# Autodesk Inventor assembly: Assembly_v2
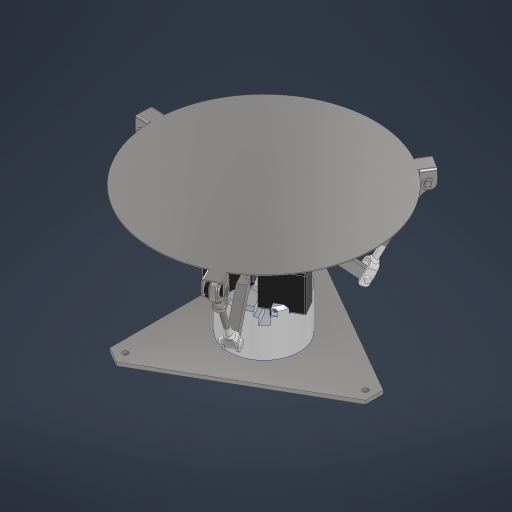
[picture p0: Inventor's stored thumbnail of the model, 512x512]
Saved by Autodesk Inventor 2023 (Build 270158000, 158)
## iProperties
Created: 2023-02-25
Part Number: Assembly_v2
Document SubType Name: Assembly
Designer: roota
Mass: 2505.51 g
Surface Area: 3613.46 cm^2
Volume: 474.073 cm^3
Density: 5.28507 g/cm^3
Author: roota
## Documents named in this file (18)
- D:\GitHub\NTUST-Mechanical-Design\Ball stabilization mechanism\3D CAD files\Mechanical Part CAD files\Assemblies\Assembly_v2.iam
- D:\GitHub\NTUST-Mechanical-Design\Ball stabilization mechanism\3D CAD files\Mechanical Part CAD files\Static Mechanisms\BasePlate.ipt
- D:\GitHub\NTUST-Mechanical-Design\Ball stabilization mechanism\3D CAD files\Mechanical Part CAD files\Static Mechanisms\BaseSupport.ipt
- D:\GitHub\NTUST-Mechanical-Design\Ball stabilization mechanism\3D CAD files\Electrical Hardware CAD files\SERVO\LDX-335MG_Servo_15kg_cm.ipt
- D:\GitHub\NTUST-Mechanical-Design\Ball stabilization mechanism\3D CAD files\Mechanical Part CAD files\Static Mechanisms\ServoCap V2.ipt
- C:\Users\roota\Documents\Inventor\Content Center Files\R2023\en-US\ISO 10642(2)\ISO 10642  - M8  x  80.ipt
- C:\Users\roota\Documents\Inventor\Content Center Files\R2023\en-US\ISO 10642(2)\ISO 10642  - M5  x  12.ipt
- C:\Users\roota\Documents\Inventor\Content Center Files\R2023\en-US\ISO 4762(2)\ISO 4762 - M5 x 12ISO.ipt
- C:\Users\roota\Documents\Inventor\Content Center Files\R2023\en-US\BS EN ISO 4026\BS EN ISO 4168 - M3 x 6(2).ipt
- D:\GitHub\NTUST-Mechanical-Design\Ball stabilization mechanism\3D CAD files\Electrical Hardware CAD files\SERVO\ServoDrive.ipt
- D:\GitHub\NTUST-Mechanical-Design\Ball stabilization mechanism\3D CAD files\Mechanical Part CAD files\Dynamic Mechanisms\Servo_Strut_v2.ipt
- D:\GitHub\NTUST-Mechanical-Design\Ball stabilization mechanism\3D CAD files\Mechanical Part CAD files\Hardware Parts\M6x1 Welded thread fork\M6x1 Welded thread fork.ipt
- D:\GitHub\NTUST-Mechanical-Design\Ball stabilization mechanism\3D CAD files\Mechanical Part CAD files\Hardware Parts\SELF-LUBRIFICATING ROD END\End_6mm.ipt
- D:\GitHub\NTUST-Mechanical-Design\Ball stabilization mechanism\3D CAD files\Mechanical Part CAD files\Hardware Parts\SELF-LUBRIFICATING ROD END\Ball_6mm_male.ipt
- D:\GitHub\NTUST-Mechanical-Design\Ball stabilization mechanism\3D CAD files\Mechanical Part CAD files\Static Mechanisms\rod pin.ipt
- C:\Users\roota\Documents\Inventor\Content Center Files\R2023\en-US\JIS B 2804 E\_JIS B 2804 E - 5 - 6.ipt
- D:\GitHub\NTUST-Mechanical-Design\Ball stabilization mechanism\3D CAD files\Mechanical Part CAD files\Static Mechanisms\4mm spacer.ipt
- D:\GitHub\NTUST-Mechanical-Design\Ball stabilization mechanism\3D CAD files\Mechanical Part CAD files\Static Mechanisms\BalancePlate.ipt
## Components (51 placed, 17 different names)
1. BasePlate:1 — Mate:46, Mate:47, Mate:48, Mate:49, Mate:50, Mate:51, Mate:63, Mate:64, Mate:65, Mate:66
2. BaseSupport:1 — Mate:49, Mate:50, Mate:51, Mate:52, Mate:53, Mate:54, Mate:55, Mate:56, Mate:57, Mate:58, Mate:59, Mate:60, Mate:67, Mate:68, Mate:69
3. LDX-335MG_Servo_15kg_cm:1 — Mate:52, Mate:53, Mate:54, Mate:61, Insert:1, Insert:2, Insert:9
4. LDX-335MG_Servo_15kg_cm:2 — Mate:55, Mate:59, Mate:60, Insert:3, Insert:4, Insert:7
5. LDX-335MG_Servo_15kg_cm:3 — Mate:56, Mate:57, Mate:58, Insert:5, Insert:6, Insert:8
6. ServoCap V2:1 — Mate:61, Mate:62, Mate:70, Mate:82
7. DIN EN ISO 10642 M8  x  80:1 — Mate:62
8. DIN EN ISO 10642 M5  x  12:1 — Mate:63
9. DIN EN ISO 10642 M5  x  12:2 — Mate:64
10. DIN EN ISO 10642 M5  x  12:3 — Mate:65
11. DIN EN ISO 10642 M5  x  12:4 — Mate:66
12. ISO 4762 M5 x 12:1 — Insert:1
13. ISO 4762 M5 x 12:2 — Insert:2
14. ISO 4762 M5 x 12:3 — Insert:3
15. ISO 4762 M5 x 12:4 — Insert:4, Mate:70
16. ISO 4762 M5 x 12:5 — Insert:5
17. ISO 4762 M5 x 12:6 — Insert:6
18. BS EN ISO 4026 - Metric M3 x 6:1 — Mate:67
19. BS EN ISO 4026 - Metric M3 x 6:2 — Mate:68
20. BS EN ISO 4026 - Metric M3 x 6:3 — Mate:69
21. ServoDrive:1 — Insert:7, Insert:10
22. ServoDrive:2 — Insert:8, Insert:11
23. ServoDrive:3 — Insert:9, Insert:12
24. Servo_Strut_v2:1 — Insert:10, Insert:13
25. Servo_Strut_v2:2 — Insert:11, Insert:14
26. Servo_Strut_v2:3 — Insert:12, Insert:15
27. M6x1 Welded thread fork:1 — Insert:13, Insert:16, Angle:1
28. M6x1 Welded thread fork:2 — Insert:14, Insert:18, Angle:2
29. M6x1 Welded thread fork:3 — Insert:15, Insert:17, Angle:3
30. End_6mm:1 — Insert:16, Angle:1, Tangent:3
31. End_6mm:2 — Insert:17, Angle:3, Tangent:1
32. End_6mm:3 — Insert:18, Angle:2, Tangent:2
33. Ball_6mm_male:1 — Tangent:1, Insert:25, Insert:26
34. Ball_6mm_male:2 — Tangent:2, Insert:29, Insert:30
35. Ball_6mm_male:3 — Tangent:3, Insert:27, Insert:28
36. rod pin:1 — Insert:23, Insert:24, Mate:71, Mate:74
37. rod pin:2 — Insert:19, Insert:20, Mate:72
38. rod pin:3 — Insert:21, Insert:22, Mate:73
39. JIS B 2804 E 5:1 — Insert:19
40. JIS B 2804 E 5:2 — Insert:20, Mate:78
41. JIS B 2804 E 5:3 — Insert:21, Mate:81
42. JIS B 2804 E 5:4 — Insert:22
43. JIS B 2804 E 5:5 — Insert:23
44. JIS B 2804 E 5:6 — Insert:24
45. 4mm spacer:1 — Insert:25, Mate:71, Mate:75
46. 4mm spacer:2 — Insert:26
47. 4mm spacer:3 — Insert:27, Mate:73, Mate:79
48. 4mm spacer:4 — Insert:28, Mate:80
49. 4mm spacer:5 — Insert:29, Mate:76, Mate:77
50. 4mm spacer:6 — Insert:30, Mate:72
51. BalancePlate:1 — Mate:74, Mate:75, Mate:76, Mate:77, Mate:78, Mate:79, Mate:80, Mate:81, Mate:82
## Relationships (73: Mate 37, Insert 30, Angle 3, Tangent 3)
- Mate:46: BasePlate:1
- Mate:47: BasePlate:1
- Mate:48: BasePlate:1
- Mate:49: BasePlate:1 ↔ BaseSupport:1
- Mate:50: BasePlate:1 ↔ BaseSupport:1
- Mate:51: BasePlate:1 ↔ BaseSupport:1
- Mate:52: BaseSupport:1 ↔ LDX-335MG_Servo_15kg_cm:1
- Mate:53: BaseSupport:1 ↔ LDX-335MG_Servo_15kg_cm:1
- Mate:54: BaseSupport:1 ↔ LDX-335MG_Servo_15kg_cm:1
- Mate:55: BaseSupport:1 ↔ LDX-335MG_Servo_15kg_cm:2
- Mate:56: BaseSupport:1 ↔ LDX-335MG_Servo_15kg_cm:3
- Mate:57: BaseSupport:1 ↔ LDX-335MG_Servo_15kg_cm:3
- Mate:58: BaseSupport:1 ↔ LDX-335MG_Servo_15kg_cm:3
- Mate:59: BaseSupport:1 ↔ LDX-335MG_Servo_15kg_cm:2
- Mate:60: BaseSupport:1 ↔ LDX-335MG_Servo_15kg_cm:2
- Mate:61: LDX-335MG_Servo_15kg_cm:1 ↔ ServoCap V2:1
- Mate:62: ServoCap V2:1 ↔ DIN EN ISO 10642 M8  x  80:1
- Mate:63: BasePlate:1 ↔ DIN EN ISO 10642 M5  x  12:1
- Mate:64: BasePlate:1 ↔ DIN EN ISO 10642 M5  x  12:2
- Mate:65: BasePlate:1 ↔ DIN EN ISO 10642 M5  x  12:3
- Mate:66: BasePlate:1 ↔ DIN EN ISO 10642 M5  x  12:4
- Insert:1: LDX-335MG_Servo_15kg_cm:1 ↔ ISO 4762 M5 x 12:1
- Insert:2: LDX-335MG_Servo_15kg_cm:1 ↔ ISO 4762 M5 x 12:2
- Insert:3: LDX-335MG_Servo_15kg_cm:2 ↔ ISO 4762 M5 x 12:3
- Insert:4: LDX-335MG_Servo_15kg_cm:2 ↔ ISO 4762 M5 x 12:4
- Insert:5: LDX-335MG_Servo_15kg_cm:3 ↔ ISO 4762 M5 x 12:5
- Insert:6: LDX-335MG_Servo_15kg_cm:3 ↔ ISO 4762 M5 x 12:6
- Mate:67: BaseSupport:1 ↔ BS EN ISO 4026 - Metric M3 x 6:1
- Mate:68: BaseSupport:1 ↔ BS EN ISO 4026 - Metric M3 x 6:2
- Mate:69: BaseSupport:1 ↔ BS EN ISO 4026 - Metric M3 x 6:3
- Mate:70: ServoCap V2:1 ↔ ISO 4762 M5 x 12:4
- Insert:7: LDX-335MG_Servo_15kg_cm:2 ↔ ServoDrive:1
- Insert:8: LDX-335MG_Servo_15kg_cm:3 ↔ ServoDrive:2
- Insert:9: LDX-335MG_Servo_15kg_cm:1 ↔ ServoDrive:3
- Insert:10: ServoDrive:1 ↔ Servo_Strut_v2:1
- Insert:11: ServoDrive:2 ↔ Servo_Strut_v2:2
- Insert:12: ServoDrive:3 ↔ Servo_Strut_v2:3
- Insert:13: Servo_Strut_v2:1 ↔ M6x1 Welded thread fork:1
- Insert:14: Servo_Strut_v2:2 ↔ M6x1 Welded thread fork:2
- Insert:15: Servo_Strut_v2:3 ↔ M6x1 Welded thread fork:3
- Insert:16 (-8 mm): M6x1 Welded thread fork:1 ↔ End_6mm:1
- Insert:17 (-8 mm): M6x1 Welded thread fork:3 ↔ End_6mm:2
- Insert:18 (-8 mm): M6x1 Welded thread fork:2 ↔ End_6mm:3
- Angle:1 (0 deg): M6x1 Welded thread fork:1 ↔ End_6mm:1
- Angle:2 (0 deg): M6x1 Welded thread fork:2 ↔ End_6mm:3
- Angle:3 (0 deg): M6x1 Welded thread fork:3 ↔ End_6mm:2
- Tangent:1: End_6mm:2 ↔ Ball_6mm_male:1
- Tangent:2: End_6mm:3 ↔ Ball_6mm_male:2
- Tangent:3: End_6mm:1 ↔ Ball_6mm_male:3
- Insert:19: rod pin:2 ↔ JIS B 2804 E 5:1
- Insert:20: rod pin:2 ↔ JIS B 2804 E 5:2
- Insert:21: rod pin:3 ↔ JIS B 2804 E 5:3
- Insert:22: rod pin:3 ↔ JIS B 2804 E 5:4
- Insert:23: rod pin:1 ↔ JIS B 2804 E 5:5
- Insert:24: rod pin:1 ↔ JIS B 2804 E 5:6
- Insert:25: Ball_6mm_male:1 ↔ 4mm spacer:1
- Insert:26: Ball_6mm_male:1 ↔ 4mm spacer:2
- Insert:27: Ball_6mm_male:3 ↔ 4mm spacer:3
- Insert:28: Ball_6mm_male:3 ↔ 4mm spacer:4
- Insert:29: Ball_6mm_male:2 ↔ 4mm spacer:5
- Insert:30: Ball_6mm_male:2 ↔ 4mm spacer:6
- Mate:71: rod pin:1 ↔ 4mm spacer:1
- Mate:72: rod pin:2 ↔ 4mm spacer:6
- Mate:73: rod pin:3 ↔ 4mm spacer:3
- Mate:74: rod pin:1 ↔ BalancePlate:1
- Mate:75: 4mm spacer:1 ↔ BalancePlate:1
- Mate:76: 4mm spacer:5 ↔ BalancePlate:1
- Mate:77: 4mm spacer:5 ↔ BalancePlate:1
- Mate:78: JIS B 2804 E 5:2 ↔ BalancePlate:1
- Mate:79: 4mm spacer:3 ↔ BalancePlate:1
- Mate:80: 4mm spacer:4 ↔ BalancePlate:1
- Mate:81: JIS B 2804 E 5:3 ↔ BalancePlate:1
- Mate:82 (60 mm): ServoCap V2:1 ↔ BalancePlate:1
## Named parameters: AngleX = 5 deg, AngleY = 5 deg
